# Autodesk Inventor assembly: jig
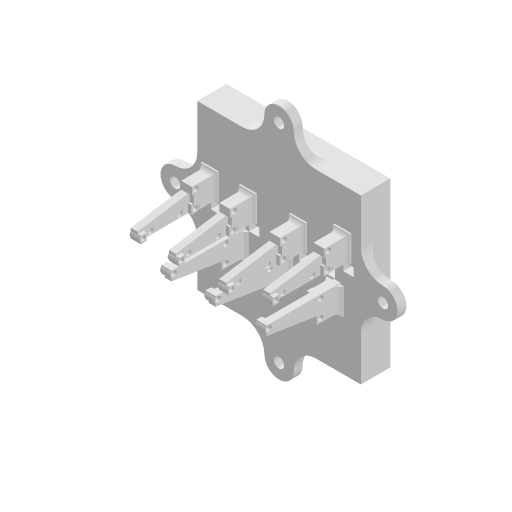
[picture p0: Inventor's stored thumbnail of the model, 512x512]
Saved by Autodesk Inventor 2023 (Build 270158030, 158C)
## iProperties
Created: 2022-08-19
Part Number: jig
Document SubType Name: Assembly
Designer: James
Author: James
## Documents named in this file (3)
- E:\OneDrive - University College London\Activation of Metasurface\Ben Motors\SSM_assembly\jig.iam
- E:\OneDrive - University College London\Activation of Metasurface\Ben Motors\SSM_assembly\frame.ipt
- E:\OneDrive - University College London\Activation of Metasurface\Ben Motors\SSM_assembly\MotorAP.ipt
## Components (8 placed, 2 different names)
1. frame:1 — Mate:1, Mate:2, Mate:3, Mate:4, Flush:1, Mate:5, Mate:6, Mate:7, Mate:8, Mate:9, Mate:10, Flush:2, Flush:3, Flush:4, Flush:5, Flush:6, Mate:11, Mate:12, Mate:13, Mate:14, Mate:15
2. MotorAP:1 — Mate:1, Mate:2, Mate:3
3. MotorAP:2 — Mate:4, Flush:1, Mate:5
4. MotorAP:3 — Mate:6, Flush:2, Mate:11
5. MotorAP:4 — Mate:7, Flush:3, Mate:15
6. MotorAP:5 — Mate:8, Flush:4, Mate:12
7. MotorAP:6 — Mate:10, Flush:6, Mate:13
8. MotorAP:7 — Mate:9, Flush:5, Mate:14
## Relationships (21: Mate 15, Flush 6)
- Mate:1 (-6.338 mm): frame:1 ↔ MotorAP:1
- Mate:2 (-19.405 mm): frame:1 ↔ MotorAP:1
- Mate:3: frame:1 ↔ MotorAP:1
- Mate:4: frame:1 ↔ MotorAP:2
- Flush:1 (4.294 mm): frame:1 ↔ MotorAP:2
- Mate:5 (-15.118 mm): frame:1 ↔ MotorAP:2
- Mate:6: frame:1 ↔ MotorAP:3
- Mate:7: frame:1 ↔ MotorAP:4
- Mate:8: frame:1 ↔ MotorAP:5
- Mate:9: frame:1 ↔ MotorAP:7
- Mate:10: frame:1 ↔ MotorAP:6
- Flush:2 (13.069 mm): frame:1 ↔ MotorAP:3
- Flush:3 (36.549 mm): frame:1 ↔ MotorAP:4
- Flush:4 (28.073 mm): frame:1 ↔ MotorAP:5
- Flush:5 (19.5 mm): frame:1 ↔ MotorAP:7
- Flush:6 (45.325 mm): frame:1 ↔ MotorAP:6
- Mate:11 (-25.25 mm): frame:1 ↔ MotorAP:3
- Mate:12 (-25.25 mm): frame:1 ↔ MotorAP:5
- Mate:13 (-25.25 mm): frame:1 ↔ MotorAP:6
- Mate:14 (-25.25 mm): frame:1 ↔ MotorAP:7
- Mate:15 (-25.25 mm): frame:1 ↔ MotorAP:4
